# Autodesk Inventor assembly: Assembly rupsbanden
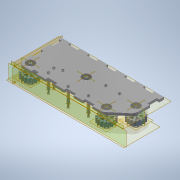
[picture p0: Inventor's stored thumbnail of the model, 180x180]
Saved by Autodesk Inventor 2021 (Build 250183000, 183)
## iProperties
Manager: PJ / DCS
Company: Emmaüs Bovenbouw Aalter
Created: 2020-11-06
Part Number: Assembly rupsbanden
Catalog Web Link: http://emmausbovenbouw.op-weg.be/
Vendor: Emmaüs Bovenbouw Aalter
Document SubType Name: Assembly
Designer: Antho
Engineer: Declercq St.
Authority: Declercq St.
Title: Algemene Projecttitel
Author: Antho
## Documents named in this file (7)
- D:\Inventor\GIP 6EM\Assembly\Assembly rupsbanden.iam
- D:\Inventor\GIP 6EM\Wielen\Rupsband.ipt
- D:\Inventor\GIP 6EM\Bevestigingen\ball bearing ISO 104 - 3 73 - 8 x 26 x 8.ipt
- D:\Inventor\GIP 6EM\waterkannon\Steun stuk.ipt
- D:\Inventor\GIP 6EM\Wielen\Wiel poging 3.ipt
- D:\Inventor\GIP 6EM\Wielen\Frame wiel binnen.ipt
- D:\Inventor\GIP 6EM\Bevestigingen\bout ISO 4762 - M4 x 16ISO.ipt
## Components (35 placed, 6 different names)
1. Rupsband:1 — Flush:1, Mate:1, Flush:2, Flush:3, Flush:4, Mate:2, Mate:3, Mate:4, Mate:5, Mate:6, Flush:5, Flush:6, Flush:7, Flush:8, Mate:11, Mate:12, Mate:13, Mate:14, Mate:15, Mate:16, Mate:17, Mate:18, Mate:19, Mate:20, Mate:21, Mate:22, Mate:37, Mate:38, Mate:39, Mate:40, Mate:41, Mate:42, Mate:43
2. ISO 104 (Single Direction) 3 73 - 8 x 26 x 8:1 — Flush:1, Mate:1, Mate:7
3. ISO 104 (Single Direction) 3 73 - 8 x 26 x 8:2 — Flush:4, Mate:4, Mate:10
4. ISO 104 (Single Direction) 3 73 - 8 x 26 x 8:3 — Flush:3, Mate:3, Mate:9
5. ISO 104 (Single Direction) 3 73 - 8 x 26 x 8:4 — Flush:2, Mate:2, Mate:8
6. Steun stuk:1 — Mate:5, Mate:6, Mate:34
7. Wiel poging 3:1 — Flush:5, Mate:7, Mate:29
8. Wiel poging 3:2 — Flush:6, Mate:8
9. Wiel poging 3:3 — Flush:7, Mate:9
10. Wiel poging 3:4 — Flush:8, Mate:10, Mate:28
11. Steun stuk:2 — Mate:14, Mate:22, Mate:23, Mate:32
12. Steun stuk:3 — Mate:16, Mate:20, Mate:30
13. Steun stuk:4 — Mate:15, Mate:18, Mate:35
14. Steun stuk:5 — Mate:12, Mate:21, Mate:33
15. Steun stuk:6 — Mate:13, Mate:19, Mate:31
16. Steun stuk:7 — Mate:11, Mate:17, Mate:36
17. Frame wiel binnen:1 — Mate:23, Flush:9, Flush:10, Flush:11, Flush:12, Mate:24, Mate:25, Mate:26, Mate:27, Mate:46, Mate:47, Mate:48, Mate:49, Mate:50, Mate:51, Mate:52, Mate:53, Mate:54, Mate:55, Mate:56, Mate:57, Mate:58, Mate:59
18. ISO 104 (Single Direction) 3 73 - 8 x 26 x 8:5 — Flush:9, Mate:24, Mate:28
19. ISO 104 (Single Direction) 3 73 - 8 x 26 x 8:6 — Flush:10, Mate:27, Mate:29
20. ISO 104 (Single Direction) 3 73 - 8 x 26 x 8:7 — Flush:11, Mate:26
21. ISO 104 (Single Direction) 3 73 - 8 x 26 x 8:8 — Flush:12, Mate:25
22. ISO 4762 M4 x 16:1 — Mate:32, Mate:39
23. ISO 4762 M4 x 16:2 — Mate:30, Mate:38
24. ISO 4762 M4 x 16:3 — Mate:33, Mate:37
25. ISO 4762 M4 x 16:4 — Mate:36, Mate:43
26. ISO 4762 M4 x 16:5 — Mate:34, Mate:41
27. ISO 4762 M4 x 16:6 — Mate:35, Mate:42
28. ISO 4762 M4 x 16:7 — Mate:31, Mate:40
29. ISO 4762 M4 x 16:8 — Mate:52, Mate:59
30. ISO 4762 M4 x 16:9 — Mate:47, Mate:53
31. ISO 4762 M4 x 16:10 — Mate:49, Mate:56
32. ISO 4762 M4 x 16:11 — Mate:46, Mate:55
33. ISO 4762 M4 x 16:12 — Mate:50, Mate:57
34. ISO 4762 M4 x 16:13 — Mate:51, Mate:58
35. ISO 4762 M4 x 16:14 — Mate:48, Mate:54
## Relationships (69: Mate 57, Flush 12)
- Flush:1: Rupsband:1 ↔ ISO 104 (Single Direction) 3 73 - 8 x 26 x 8:1
- Mate:1: Rupsband:1 ↔ ISO 104 (Single Direction) 3 73 - 8 x 26 x 8:1
- Flush:2: Rupsband:1 ↔ ISO 104 (Single Direction) 3 73 - 8 x 26 x 8:4
- Flush:3: Rupsband:1 ↔ ISO 104 (Single Direction) 3 73 - 8 x 26 x 8:3
- Flush:4: Rupsband:1 ↔ ISO 104 (Single Direction) 3 73 - 8 x 26 x 8:2
- Mate:2: Rupsband:1 ↔ ISO 104 (Single Direction) 3 73 - 8 x 26 x 8:4
- Mate:3: Rupsband:1 ↔ ISO 104 (Single Direction) 3 73 - 8 x 26 x 8:3
- Mate:4: Rupsband:1 ↔ ISO 104 (Single Direction) 3 73 - 8 x 26 x 8:2
- Mate:5: Rupsband:1 ↔ Steun stuk:1
- Mate:6: Rupsband:1 ↔ Steun stuk:1
- Flush:5: Rupsband:1 ↔ Wiel poging 3:1
- Mate:7: ISO 104 (Single Direction) 3 73 - 8 x 26 x 8:1 ↔ Wiel poging 3:1
- Flush:6: Rupsband:1 ↔ Wiel poging 3:2
- Flush:7: Rupsband:1 ↔ Wiel poging 3:3
- Flush:8: Rupsband:1 ↔ Wiel poging 3:4
- Mate:8: ISO 104 (Single Direction) 3 73 - 8 x 26 x 8:4 ↔ Wiel poging 3:2
- Mate:9: ISO 104 (Single Direction) 3 73 - 8 x 26 x 8:3 ↔ Wiel poging 3:3
- Mate:10: ISO 104 (Single Direction) 3 73 - 8 x 26 x 8:2 ↔ Wiel poging 3:4
- Mate:11: Rupsband:1 ↔ Steun stuk:7
- Mate:12: Rupsband:1 ↔ Steun stuk:5
- Mate:13: Rupsband:1 ↔ Steun stuk:6
- Mate:14: Rupsband:1 ↔ Steun stuk:2
- Mate:15: Rupsband:1 ↔ Steun stuk:4
- Mate:16: Rupsband:1 ↔ Steun stuk:3
- Mate:17: Rupsband:1 ↔ Steun stuk:7
- Mate:18: Rupsband:1 ↔ Steun stuk:4
- Mate:19: Rupsband:1 ↔ Steun stuk:6
- Mate:20: Rupsband:1 ↔ Steun stuk:3
- Mate:21: Rupsband:1 ↔ Steun stuk:5
- Mate:22: Rupsband:1 ↔ Steun stuk:2
- Mate:23: Steun stuk:2 ↔ Frame wiel binnen:1
- Flush:9: Frame wiel binnen:1 ↔ ISO 104 (Single Direction) 3 73 - 8 x 26 x 8:5
- Flush:10: Frame wiel binnen:1 ↔ ISO 104 (Single Direction) 3 73 - 8 x 26 x 8:6
- Flush:11: Frame wiel binnen:1 ↔ ISO 104 (Single Direction) 3 73 - 8 x 26 x 8:7
- Flush:12: Frame wiel binnen:1 ↔ ISO 104 (Single Direction) 3 73 - 8 x 26 x 8:8
- Mate:24: Frame wiel binnen:1 ↔ ISO 104 (Single Direction) 3 73 - 8 x 26 x 8:5
- Mate:25: Frame wiel binnen:1 ↔ ISO 104 (Single Direction) 3 73 - 8 x 26 x 8:8
- Mate:26: Frame wiel binnen:1 ↔ ISO 104 (Single Direction) 3 73 - 8 x 26 x 8:7
- Mate:27: Frame wiel binnen:1 ↔ ISO 104 (Single Direction) 3 73 - 8 x 26 x 8:6
- Mate:28: Wiel poging 3:4 ↔ ISO 104 (Single Direction) 3 73 - 8 x 26 x 8:5
- Mate:29: Wiel poging 3:1 ↔ ISO 104 (Single Direction) 3 73 - 8 x 26 x 8:6
- Mate:30: Steun stuk:3 ↔ ISO 4762 M4 x 16:2
- Mate:31: Steun stuk:6 ↔ ISO 4762 M4 x 16:7
- Mate:32: Steun stuk:2 ↔ ISO 4762 M4 x 16:1
- Mate:33: Steun stuk:5 ↔ ISO 4762 M4 x 16:3
- Mate:34: Steun stuk:1 ↔ ISO 4762 M4 x 16:5
- Mate:35: Steun stuk:4 ↔ ISO 4762 M4 x 16:6
- Mate:36: Steun stuk:7 ↔ ISO 4762 M4 x 16:4
- Mate:37: Rupsband:1 ↔ ISO 4762 M4 x 16:3
- Mate:38: Rupsband:1 ↔ ISO 4762 M4 x 16:2
- Mate:39: Rupsband:1 ↔ ISO 4762 M4 x 16:1
- Mate:40: Rupsband:1 ↔ ISO 4762 M4 x 16:7
- Mate:41: Rupsband:1 ↔ ISO 4762 M4 x 16:5
- Mate:42: Rupsband:1 ↔ ISO 4762 M4 x 16:6
- Mate:43: Rupsband:1 ↔ ISO 4762 M4 x 16:4
- Mate:46: Frame wiel binnen:1 ↔ ISO 4762 M4 x 16:11
- Mate:47: Frame wiel binnen:1 ↔ ISO 4762 M4 x 16:9
- Mate:48: Frame wiel binnen:1 ↔ ISO 4762 M4 x 16:14
- Mate:49: Frame wiel binnen:1 ↔ ISO 4762 M4 x 16:10
- Mate:50: Frame wiel binnen:1 ↔ ISO 4762 M4 x 16:12
- Mate:51: Frame wiel binnen:1 ↔ ISO 4762 M4 x 16:13
- Mate:52: Frame wiel binnen:1 ↔ ISO 4762 M4 x 16:8
- Mate:53: Frame wiel binnen:1 ↔ ISO 4762 M4 x 16:9
- Mate:54: Frame wiel binnen:1 ↔ ISO 4762 M4 x 16:14
- Mate:55: Frame wiel binnen:1 ↔ ISO 4762 M4 x 16:11
- Mate:56: Frame wiel binnen:1 ↔ ISO 4762 M4 x 16:10
- Mate:57: Frame wiel binnen:1 ↔ ISO 4762 M4 x 16:12
- Mate:58: Frame wiel binnen:1 ↔ ISO 4762 M4 x 16:13
- Mate:59: Frame wiel binnen:1 ↔ ISO 4762 M4 x 16:8
